# Autodesk Inventor assembly: Battery holder assembly
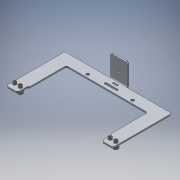
[picture p0: Inventor's stored thumbnail of the model, 180x180]
Saved by Autodesk Inventor 2018 (Build 220112000, 112)
## iProperties
Created: 2020-01-28
Part Number: Battery holder assembly
Document SubType Name: Assembly
Designer: maste
Author: maste
## Documents named in this file (6)
- C:\Users\maste\OneDrive\Documents\GitHub\2020CAD\Drivebase AM14U1\Part Files\Battery holder assembly.iam
- C:\Users\maste\OneDrive\Documents\GitHub\2020CAD\Drivebase AM14U1\Part Files\am-3958 AM14U4 Vertical Battery Mount C Plate.ipt
- C:\Users\maste\OneDrive\Documents\GitHub\2020CAD\Drivebase AM14U1\Part Files\3.375in Churro.ipt
- C:\Users\maste\OneDrive\Documents\GitHub\2020CAD\Drivebase AM14U1\Part Files\Bolts\96024A420_THREAD-CUTTING SCREW.ipt
- C:\Users\maste\OneDrive\Documents\GitHub\2020CAD\Drivebase AM14U1\Part Files\Bolts\92196A269_18-8 STAINLESS STEEL SOCKET HEAD CAP SCREW.ipt
- C:\Users\maste\OneDrive\Documents\GitHub\2020CAD\Drivebase AM14U1\Part Files\Locknuts\91831A411_TYPE 18-8 STAINLESS STL NYLON-INSERT LOCKNUT.ipt
## Components (13 placed, 5 different names)
1. am-3958 AM14U4 Vertical Battery Mount C Plate:1 — Mate:1, Mate:2, Mate:3, Mate:4, Rotation:1, Rotation:2, Mate:13, Mate:14, Mate:15, Mate:16, Rotation:7, Rotation:8, Mate:17, Mate:18, Mate:19, Mate:20, Mate:21, Mate:22, Mate:23, Mate:24, Mate:25, Mate:27, Mate:29, Mate:31, Rotation:9, Rotation:10, Rotation:11, Rotation:12, Rotation:13, Rotation:14, Rotation:15, Rotation:16
2. 3.375in Churro:1 — Mate:1, Mate:2, Rotation:2
3. 3.375in Churro:2 — Mate:3, Mate:4, Rotation:1
4. 96024A420_THREAD-CUTTING SCREW:1 — Mate:13, Mate:15, Rotation:8
5. 96024A420_THREAD-CUTTING SCREW:2 — Mate:14, Mate:16, Rotation:7
6. 92196A269_18-8 STAINLESS STEEL SOCKET HEAD CAP SCREW:1 — Mate:17, Mate:24, Mate:26, Rotation:13
7. 92196A269_18-8 STAINLESS STEEL SOCKET HEAD CAP SCREW:2 — Mate:18, Mate:23, Mate:28, Rotation:14
8. 92196A269_18-8 STAINLESS STEEL SOCKET HEAD CAP SCREW:3 — Mate:19, Mate:21, Mate:30, Rotation:15
9. 92196A269_18-8 STAINLESS STEEL SOCKET HEAD CAP SCREW:4 — Mate:20, Mate:22, Mate:32, Rotation:16
10. 91831A411_TYPE 18-8 STAINLESS STL NYLON-INSERT LOCKNUT:1 — Mate:29, Mate:30, Rotation:10
11. 91831A411_TYPE 18-8 STAINLESS STL NYLON-INSERT LOCKNUT:2 — Mate:31, Mate:32, Rotation:9
12. 91831A411_TYPE 18-8 STAINLESS STL NYLON-INSERT LOCKNUT:3 — Mate:27, Mate:28, Rotation:11
13. 91831A411_TYPE 18-8 STAINLESS STL NYLON-INSERT LOCKNUT:4 — Mate:25, Mate:26, Rotation:12
## Relationships (36: Mate 24, RelateRotation 12)
- Mate:1: am-3958 AM14U4 Vertical Battery Mount C Plate:1 ↔ 3.375in Churro:1
- Mate:2: am-3958 AM14U4 Vertical Battery Mount C Plate:1 ↔ 3.375in Churro:1
- Mate:3: am-3958 AM14U4 Vertical Battery Mount C Plate:1 ↔ 3.375in Churro:2
- Mate:4: am-3958 AM14U4 Vertical Battery Mount C Plate:1 ↔ 3.375in Churro:2
- Rotation:1 [RelateRotation] (1 ul): am-3958 AM14U4 Vertical Battery Mount C Plate:1 ↔ 3.375in Churro:2
- Rotation:2 [RelateRotation] (1 ul): am-3958 AM14U4 Vertical Battery Mount C Plate:1 ↔ 3.375in Churro:1
- Mate:13: am-3958 AM14U4 Vertical Battery Mount C Plate:1 ↔ 96024A420_THREAD-CUTTING SCREW:1
- Mate:14: am-3958 AM14U4 Vertical Battery Mount C Plate:1 ↔ 96024A420_THREAD-CUTTING SCREW:2
- Mate:15: am-3958 AM14U4 Vertical Battery Mount C Plate:1 ↔ 96024A420_THREAD-CUTTING SCREW:1
- Mate:16: am-3958 AM14U4 Vertical Battery Mount C Plate:1 ↔ 96024A420_THREAD-CUTTING SCREW:2
- Rotation:7 [RelateRotation] (1 ul): am-3958 AM14U4 Vertical Battery Mount C Plate:1 ↔ 96024A420_THREAD-CUTTING SCREW:2
- Rotation:8 [RelateRotation] (1 ul): am-3958 AM14U4 Vertical Battery Mount C Plate:1 ↔ 96024A420_THREAD-CUTTING SCREW:1
- Mate:17: am-3958 AM14U4 Vertical Battery Mount C Plate:1 ↔ 92196A269_18-8 STAINLESS STEEL SOCKET HEAD CAP SCREW:1
- Mate:18: am-3958 AM14U4 Vertical Battery Mount C Plate:1 ↔ 92196A269_18-8 STAINLESS STEEL SOCKET HEAD CAP SCREW:2
- Mate:19: am-3958 AM14U4 Vertical Battery Mount C Plate:1 ↔ 92196A269_18-8 STAINLESS STEEL SOCKET HEAD CAP SCREW:3
- Mate:20: am-3958 AM14U4 Vertical Battery Mount C Plate:1 ↔ 92196A269_18-8 STAINLESS STEEL SOCKET HEAD CAP SCREW:4
- Mate:21: am-3958 AM14U4 Vertical Battery Mount C Plate:1 ↔ 92196A269_18-8 STAINLESS STEEL SOCKET HEAD CAP SCREW:3
- Mate:22: am-3958 AM14U4 Vertical Battery Mount C Plate:1 ↔ 92196A269_18-8 STAINLESS STEEL SOCKET HEAD CAP SCREW:4
- Mate:23: am-3958 AM14U4 Vertical Battery Mount C Plate:1 ↔ 92196A269_18-8 STAINLESS STEEL SOCKET HEAD CAP SCREW:2
- Mate:24: am-3958 AM14U4 Vertical Battery Mount C Plate:1 ↔ 92196A269_18-8 STAINLESS STEEL SOCKET HEAD CAP SCREW:1
- Mate:25 (3.175 mm): am-3958 AM14U4 Vertical Battery Mount C Plate:1 ↔ 91831A411_TYPE 18-8 STAINLESS STL NYLON-INSERT LOCKNUT:4
- Mate:26: 92196A269_18-8 STAINLESS STEEL SOCKET HEAD CAP SCREW:1 ↔ 91831A411_TYPE 18-8 STAINLESS STL NYLON-INSERT LOCKNUT:4
- Mate:27 (3.175 mm): am-3958 AM14U4 Vertical Battery Mount C Plate:1 ↔ 91831A411_TYPE 18-8 STAINLESS STL NYLON-INSERT LOCKNUT:3
- Mate:28: 92196A269_18-8 STAINLESS STEEL SOCKET HEAD CAP SCREW:2 ↔ 91831A411_TYPE 18-8 STAINLESS STL NYLON-INSERT LOCKNUT:3
- Mate:29 (3.175 mm): am-3958 AM14U4 Vertical Battery Mount C Plate:1 ↔ 91831A411_TYPE 18-8 STAINLESS STL NYLON-INSERT LOCKNUT:1
- Mate:30: 92196A269_18-8 STAINLESS STEEL SOCKET HEAD CAP SCREW:3 ↔ 91831A411_TYPE 18-8 STAINLESS STL NYLON-INSERT LOCKNUT:1
- Mate:31 (3.175 mm): am-3958 AM14U4 Vertical Battery Mount C Plate:1 ↔ 91831A411_TYPE 18-8 STAINLESS STL NYLON-INSERT LOCKNUT:2
- Mate:32: 92196A269_18-8 STAINLESS STEEL SOCKET HEAD CAP SCREW:4 ↔ 91831A411_TYPE 18-8 STAINLESS STL NYLON-INSERT LOCKNUT:2
- Rotation:9 [RelateRotation] (1 ul): am-3958 AM14U4 Vertical Battery Mount C Plate:1 ↔ 91831A411_TYPE 18-8 STAINLESS STL NYLON-INSERT LOCKNUT:2
- Rotation:10 [RelateRotation] (1 ul): am-3958 AM14U4 Vertical Battery Mount C Plate:1 ↔ 91831A411_TYPE 18-8 STAINLESS STL NYLON-INSERT LOCKNUT:1
- Rotation:11 [RelateRotation] (1 ul): am-3958 AM14U4 Vertical Battery Mount C Plate:1 ↔ 91831A411_TYPE 18-8 STAINLESS STL NYLON-INSERT LOCKNUT:3
- Rotation:12 [RelateRotation] (1 ul): am-3958 AM14U4 Vertical Battery Mount C Plate:1 ↔ 91831A411_TYPE 18-8 STAINLESS STL NYLON-INSERT LOCKNUT:4
- Rotation:13 [RelateRotation] (1 ul): am-3958 AM14U4 Vertical Battery Mount C Plate:1 ↔ 92196A269_18-8 STAINLESS STEEL SOCKET HEAD CAP SCREW:1
- Rotation:14 [RelateRotation] (1 ul): am-3958 AM14U4 Vertical Battery Mount C Plate:1 ↔ 92196A269_18-8 STAINLESS STEEL SOCKET HEAD CAP SCREW:2
- Rotation:15 [RelateRotation] (1 ul): am-3958 AM14U4 Vertical Battery Mount C Plate:1 ↔ 92196A269_18-8 STAINLESS STEEL SOCKET HEAD CAP SCREW:3
- Rotation:16 [RelateRotation] (1 ul): am-3958 AM14U4 Vertical Battery Mount C Plate:1 ↔ 92196A269_18-8 STAINLESS STEEL SOCKET HEAD CAP SCREW:4
